# Autodesk Inventor assembly: Assembly
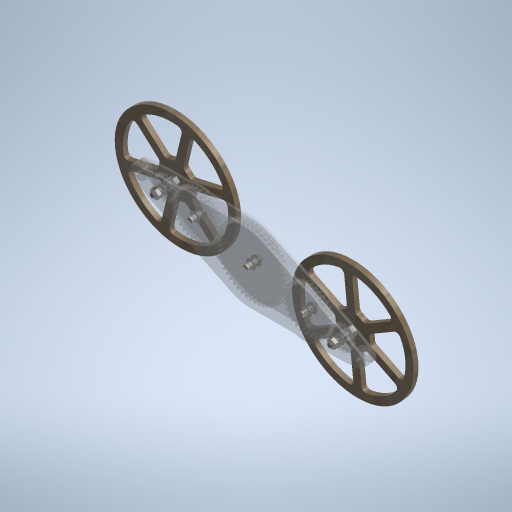
[picture p0: Inventor's stored thumbnail of the model, 512x512]
Saved by Autodesk Inventor 2023 (Build 270158000, 158)
## iProperties
Part Number: Assembly
Document SubType Name: Assembly
Designer: Ronan
Author: Ronan
## Documents named in this file (8)
- D:\Libraries\Documents\2023-FYP\Inventor\Assembly.iam
- D:\Libraries\Documents\2023-FYP\Inventor\frame.ipt
- D:\Libraries\Documents\2023-FYP\Inventor\Shaft2.ipt
- D:\Libraries\Documents\2023-FYP\Inventor\Assembly\Design Accelerator\Spur Gears3.iam
- D:\Libraries\Documents\2023-FYP\Inventor\standoff1.ipt
- D:\Libraries\Documents\2023-FYP\Inventor\wheel shaft.iam
- D:\Libraries\Documents\2023-FYP\Inventor\Assembly\Design Accelerator\Spur Gear14.ipt
- D:\Libraries\Documents\2023-FYP\Inventor\M5-washer.ipt
## Components (17 placed, 7 different names)
1. frame:1 — Rotational:1, Rotational:2, Cylindrical:1, Mate:11, Mate:12, Mate:15, Mate:17, Mate:18, Cylindrical:4, Mate:33, Mate:34
2. Shaft:2 — Rotational:1, Mate:5, Cylindrical:12
3. Shaft:3 — Rotational:2, Mate:3, Mate:7
4. Shaft:4 — Cylindrical:1, Mate:3, Rotation:1, Mate:22, Cylindrical:7
5. Spur Gears:1 [sub-assembly] — Mate:5, Mate:7, Rotation:2, Rotation:3, Mate:27, Mate:28, Mate:29, Mate:30
6. standoff1:1 — Mate:11, Mate:14, Mate:16, Mate:17, Mate:18
7. standoff1:2 — Mate:12, Mate:13, Mate:15
8. frame:2 — Mate:13, Mate:14, Mate:16, Cylindrical:2, Cylindrical:3, Cylindrical:8, Cylindrical:9, Cylindrical:10, Cylindrical:11, Mate:25, Mate:26
9. wheel shaft:1 [sub-assembly] — Cylindrical:2, Rotation:3, Mate:26
10. wheel shaft:2 [sub-assembly] — Cylindrical:3, Rotation:1, Mate:25
11. Spur Gear1:1 — Cylindrical:4, Mate:22, Rotation:2, Mate:31, Mate:32
12. M5-washer:3 — Cylindrical:7, Mate:31
13. M5-washer:4 — Cylindrical:8, Mate:32, Mate:33
14. M5-washer:5 — Cylindrical:9, Mate:29
15. M5-washer:6 — Cylindrical:10, Mate:30, Mate:34
16. M5-washer:7 — Cylindrical:11, Mate:27
17. M5-washer:8 — Cylindrical:12, Mate:28
## Relationships (37: Mate 22, CylindricalJoint 10, RelateRotation 3, RevoluteJoint 2)
- Rotational:1 [RevoluteJoint] (-4.5 mm): frame:1 ↔ Shaft:2
- Rotational:2 [RevoluteJoint] (1.5 mm): frame:1 ↔ Shaft:3
- Cylindrical:1: frame:1 ↔ Shaft:4
- Mate:3: Shaft:3 ↔ Shaft:4
- Mate:5: Shaft:2 ↔ Spur Gears:1
- Mate:7: Shaft:3 ↔ Spur Gears:1
- Mate:11: frame:1 ↔ standoff1:1
- Mate:12: frame:1 ↔ standoff1:2
- Mate:13: standoff1:2 ↔ frame:2
- Mate:14: standoff1:1 ↔ frame:2
- Mate:15: frame:1 ↔ standoff1:2
- Mate:16: standoff1:1 ↔ frame:2
- Cylindrical:2: frame:2 ↔ wheel shaft:1
- Mate:17: frame:1 ↔ standoff1:1
- Mate:18: frame:1 ↔ standoff1:1
- Cylindrical:3: frame:2 ↔ wheel shaft:2
- Rotation:1 [RelateRotation] (-0.4848 ul): Shaft:4 ↔ wheel shaft:2
- Cylindrical:4: frame:1 ↔ Spur Gear1:1
- Mate:22: Shaft:4 ↔ Spur Gear1:1
- Rotation:2 [RelateRotation] (-1.5152 ul): Spur Gears:1 ↔ Spur Gear1:1
- Rotation:3 [RelateRotation] (-0.4848 ul): Spur Gears:1 ↔ wheel shaft:1
- Cylindrical:7: Shaft:4 ↔ M5-washer:3
- Cylindrical:8: frame:2 ↔ M5-washer:4
- Cylindrical:9: frame:2 ↔ M5-washer:5
- Cylindrical:10: frame:2 ↔ M5-washer:6
- Cylindrical:11: frame:2 ↔ M5-washer:7
- Cylindrical:12: Shaft:2 ↔ M5-washer:8
- Mate:25: frame:2 ↔ wheel shaft:2
- Mate:26: frame:2 ↔ wheel shaft:1
- Mate:27: Spur Gears:1 ↔ M5-washer:7
- Mate:28: Spur Gears:1 ↔ M5-washer:8
- Mate:29: Spur Gears:1 ↔ M5-washer:5
- Mate:30: Spur Gears:1 ↔ M5-washer:6
- Mate:31: Spur Gear1:1 ↔ M5-washer:3
- Mate:32: Spur Gear1:1 ↔ M5-washer:4
- Mate:33: frame:1 ↔ M5-washer:4
- Mate:34: frame:1 ↔ M5-washer:6
